# Autodesk Inventor assembly: hip_connector_rotated
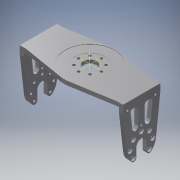
[picture p0: Inventor's stored thumbnail of the model, 180x180]
Saved by Autodesk Inventor 2018 (Build 220112000, 112)
## iProperties
Created: 2018-11-28
Part Number: hip_connector_rotated
Document SubType Name: Assembly
Designer: bitbots
Author: bitbots
## Documents named in this file (2)
- C:\Users\bitbots\Desktop\bitbots_hardware\wolfgang\assembly\body\hip_connector_rotated.iam
- C:\Users\bitbots\Desktop\bitbots_hardware\wolfgang\assembly\body\hip_connector.ipt
## Components (1 placed, 1 different names)
1. hip_connector:1 — Flush:1, Mate:1
## Relationships (2: Flush 1, Mate 1)
- Flush:1: hip_connector:1
- Mate:1: hip_connector:1
